# Autodesk Inventor assembly: led_7seg_with_sec_v3
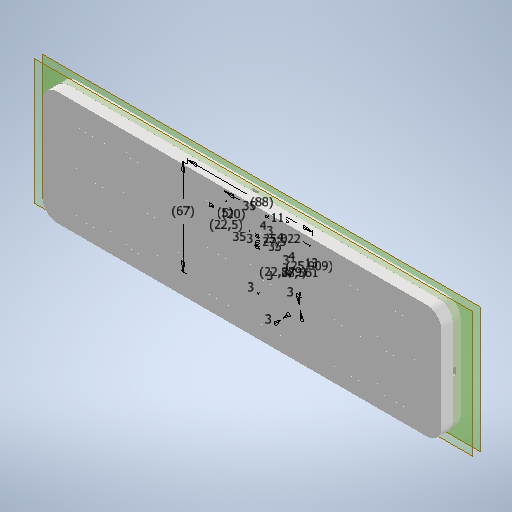
[picture p0: Inventor's stored thumbnail of the model, 512x512]
Saved by Autodesk Inventor 2026 (Build 300175000, 175)
## iProperties
Created: 2025-08-14
Part Number: led_7seg_with_sec_v3
Document SubType Name: Assembly
Designer: Korobeynikov
Author: Korobeynikov
## Documents named in this file (4)
- P:\_desktop\Inventor\led_7seg_with_sec_v3.iam
- P:\_desktop\Inventor\led 7 seg with sec v3.ipt
- P:\_desktop\Inventor\led 7 seg with sec v3 bottom.ipt
- P:\_desktop\Inventor\led 7 seg with sec v3 wall holder.ipt
## Components (3 placed, 3 different names)
1. led 7 seg with sec v3:1 — Flush:1, Flush:2
2. led 7 seg with sec v3 bottom:1 — Flush:1, Flush:2, Flush:3, Flush:4, Flush:5
3. led 7 seg with sec v3 wall holder:1 — Flush:3, Flush:4, Flush:5
## Relationships (5: Flush 5)
- Flush:1: led 7 seg with sec v3:1 ↔ led 7 seg with sec v3 bottom:1
- Flush:2: led 7 seg with sec v3:1 ↔ led 7 seg with sec v3 bottom:1
- Flush:3: led 7 seg with sec v3 bottom:1 ↔ led 7 seg with sec v3 wall holder:1
- Flush:4: led 7 seg with sec v3 bottom:1 ↔ led 7 seg with sec v3 wall holder:1
- Flush:5: led 7 seg with sec v3 bottom:1 ↔ led 7 seg with sec v3 wall holder:1
